# Autodesk Inventor assembly: Robot Chassis Half
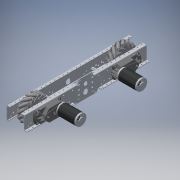
[picture p0: Inventor's stored thumbnail of the model, 180x180]
Saved by Autodesk Inventor 2017 (Build 210142000, 142)
## iProperties
Created: 2017-01-10
Part Number: Robot Chassis Half
Document SubType Name: Assembly
Designer: Roksbot
Author: Roksbot
## Documents named in this file (10)
- C:\Users\Roksbot\Documents\Inventor\2017 Robot\Robot Chassis Half.iam
- C:\Users\Roksbot\Documents\Inventor\2017 Robot\am-2952a_AM14U3_Inside_Plate.ipt
- C:\Users\Roksbot\Documents\Inventor\2017 Robot\Left-6-inch-HD-Mecanum-Wheel.ipt
- C:\Users\Roksbot\Documents\Inventor\2017 Robot\Right-6-inch-HD-Mecanum-Wheel.ipt
- C:\Users\Roksbot\Documents\Inventor\2017 Robot\3.875 Churo.ipt
- C:\Users\Roksbot\Documents\Inventor\2017 Robot\am-2951a_AM14U3_Outside_Plate.ipt
- C:\Users\Roksbot\Documents\Inventor\2017 Robot\Short Build Volume.ipt
- C:\Users\Roksbot\Documents\Inventor\2017 Robot\Tall Build Volume.ipt
- C:\Users\Roksbot\Documents\Inventor\2017 Robot\am-3230+ToughboxMicrowithFlatPlate.ipt
- C:\Users\Roksbot\Documents\Inventor\2017 Robot\am-0255+2.5inch+CIM+Motor.ipt
## Components (12 placed, 9 different names)
1. am-2952a_AM14U3_Inside_Plate:1 — Mate:1, Mate:2, Mate:4, Mate:5, Insert:1, Insert:2, Mate:6, Flush:4, Insert:4, Mate:7, Insert:5, Mate:8
2. Left-6-inch-HD-Mecanum-Wheel:1 — Flush:1, Mate:5, Fake wheel spacing
3. Right-6-inch-HD-Mecanum-Wheel:1 — Flush:1, Mate:4
4. 3.875 Churo:1 — Insert:2
5. 3.875 Churo:2 — Insert:1, Insert:3
6. am-2951a_AM14U3_Outside_Plate:1 — Mate:6, Insert:3, Flush:3, Fake wheel spacing
7. Short Build Volume:1 — Flush:3, Flush:4, Flush:5, Flush:6, Flush:7
8. Tall Build Volume:1 — Flush:5, Flush:6, Flush:7
9. am-3230+ToughboxMicrowithFlatPlate:1 — Insert:5, Mate:8, Insert:7
10. am-3230+ToughboxMicrowithFlatPlate:2 — Insert:4, Mate:7, Insert:6
11. am-0255+2.5inch+CIM+Motor:1 — Insert:6
12. am-0255+2.5inch+CIM+Motor:2 — Insert:7
## Relationships (21: Mate 8, Insert 7, Flush 6)
- Mate:1 (-254 mm): am-2952a_AM14U3_Inside_Plate:1
- Mate:2: am-2952a_AM14U3_Inside_Plate:1
- Flush:1: Left-6-inch-HD-Mecanum-Wheel:1 ↔ Right-6-inch-HD-Mecanum-Wheel:1
- Mate:4: am-2952a_AM14U3_Inside_Plate:1 ↔ Right-6-inch-HD-Mecanum-Wheel:1
- Mate:5: am-2952a_AM14U3_Inside_Plate:1 ↔ Left-6-inch-HD-Mecanum-Wheel:1
- Insert:1: am-2952a_AM14U3_Inside_Plate:1 ↔ 3.875 Churo:2
- Insert:2: am-2952a_AM14U3_Inside_Plate:1 ↔ 3.875 Churo:1
- Mate:6: am-2952a_AM14U3_Inside_Plate:1 ↔ am-2951a_AM14U3_Outside_Plate:1
- Insert:3: 3.875 Churo:2 ↔ am-2951a_AM14U3_Outside_Plate:1
- Flush:3 (-88.9 mm): am-2951a_AM14U3_Outside_Plate:1 ↔ Short Build Volume:1
- Flush:4 (-38.1 mm): am-2952a_AM14U3_Inside_Plate:1 ↔ Short Build Volume:1
- Flush:5: Short Build Volume:1 ↔ Tall Build Volume:1
- Flush:6: Short Build Volume:1 ↔ Tall Build Volume:1
- Flush:7: Short Build Volume:1 ↔ Tall Build Volume:1
- Insert:4: am-2952a_AM14U3_Inside_Plate:1 ↔ am-3230+ToughboxMicrowithFlatPlate:2
- Mate:7: am-2952a_AM14U3_Inside_Plate:1 ↔ am-3230+ToughboxMicrowithFlatPlate:2
- Insert:5: am-2952a_AM14U3_Inside_Plate:1 ↔ am-3230+ToughboxMicrowithFlatPlate:1
- Mate:8: am-2952a_AM14U3_Inside_Plate:1 ↔ am-3230+ToughboxMicrowithFlatPlate:1
- Insert:6: am-3230+ToughboxMicrowithFlatPlate:2 ↔ am-0255+2.5inch+CIM+Motor:1
- Insert:7: am-3230+ToughboxMicrowithFlatPlate:1 ↔ am-0255+2.5inch+CIM+Motor:2
- Fake wheel spacing [Mate] (12.7 mm): Left-6-inch-HD-Mecanum-Wheel:1 ↔ am-2951a_AM14U3_Outside_Plate:1
